# Autodesk Inventor assembly: StraightPumpRegion
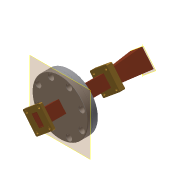
[picture p0: Inventor's stored thumbnail of the model, 180x180]
Saved by Autodesk Inventor 2015 (Build 190159000, 159)
## iProperties
Created: 2014-03-24
Part Number: StraightPumpRegion
Document SubType Name: Assembly
Designer: jad211
Author: jad211
## Documents named in this file (5)
- C:\CADFiles\EDM Machine\EDM New Pumping Region\StraightPumpRegion.iam
- C:\CADFiles\EDM Machine\EDM New Pumping Region\NewHorn.ipt
- C:\CADFiles\EDM Machine\EDM New Pumping Region\FlangedWaveguide.iam
- C:\CADFiles\EDM Machine\EDM New Pumping Region\3-38sWithWG18Hole.ipt
- C:\CADFiles\EDM Machine\EDM New Pumping Region\WG18FLANGE.ipt
## Components (4 placed, 4 different names)
1. NewHorn:1 — Angle:2, Mate:21, Flush:20, Mate:27
2. WG18FLANGE:1 — Mate:24, Mate:25, Mate:26, Mate:27
3. FlangedWaveguide:2 [sub-assembly] — Mate:21, Mate:22, Mate:23, Mate:24, Mate:25, Mate:26, Mate:28
4. 3-38sWithWG18Hole:1 — Mate:22, Mate:23, Mate:28
## Relationships (10: Mate 8, Angle 1, Flush 1)
- Angle:2 (0 deg): NewHorn:1
- Mate:21: NewHorn:1 ↔ FlangedWaveguide:2
- Flush:20 (-30 mm): NewHorn:1
- Mate:22: FlangedWaveguide:2 ↔ 3-38sWithWG18Hole:1
- Mate:23: FlangedWaveguide:2 ↔ 3-38sWithWG18Hole:1
- Mate:24: WG18FLANGE:1 ↔ FlangedWaveguide:2
- Mate:25: WG18FLANGE:1 ↔ FlangedWaveguide:2
- Mate:26: WG18FLANGE:1 ↔ FlangedWaveguide:2
- Mate:27: NewHorn:1 ↔ WG18FLANGE:1
- Mate:28 (30 mm): FlangedWaveguide:2 ↔ 3-38sWithWG18Hole:1
